# Autodesk Inventor assembly: teljes3
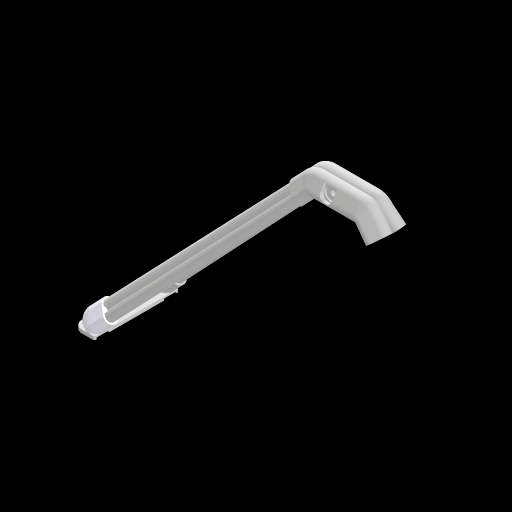
[picture p0: Inventor's stored thumbnail of the model, 512x512]
Saved by Autodesk Inventor 2023 (Build 270158000, 158)
## iProperties
Created: 2022-11-11
Part Number: teljes3
Document SubType Name: Assembly
Designer: gd1
Author: gd1
## Documents named in this file (6)
- C:\Users\gd1\3D Objects\3D nagyteherbírású híd\Híd\H-d\teljes5.iam
- C:\Users\gd1\3D Objects\3D nagyteherbírású híd\Híd\H-d\45 fok középre_talp.ipt
- C:\Users\gd1\3D Objects\3D nagyteherbírású híd\Híd\H-d\palca 325mm.ipt
- C:\Users\gd1\3D Objects\3D nagyteherbírású híd\Híd\H-d\45 fok kozepcsati.ipt.iam
- C:\Users\gd1\3D Objects\3D nagyteherbírású híd\Híd\H-d\tipli.ipt
- 45 fok kozepcsati.ipt
## Components (6 placed, 4 different names)
1. 45 fok középre_talp:1 — Rotational:1, Rotational:2
2. palca 325mm:1 — Rotational:2
3. palca 325mm:2 — Rotational:1
4. 45 fok kozepcsati.ipt:1 [sub-assembly]
5. tipli:1
6. tipli:2
## Relationships (2: RevoluteJoint 2)
- Rotational:1 [RevoluteJoint]: 45 fok középre_talp:1 ↔ palca 325mm:2
- Rotational:2 [RevoluteJoint]: 45 fok középre_talp:1 ↔ palca 325mm:1
